# Autodesk Inventor assembly: Idler Right
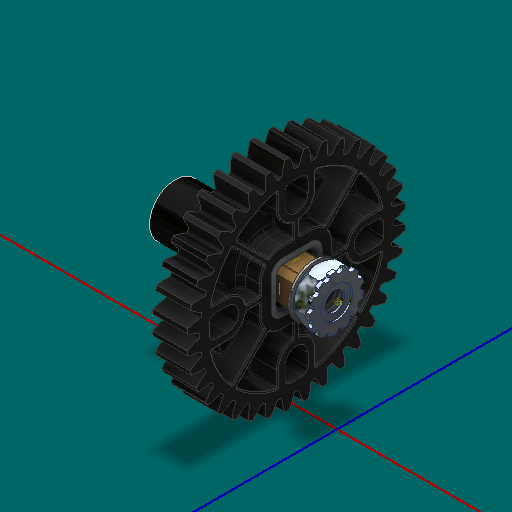
[picture p0: Inventor's stored thumbnail of the model, 512x512]
Saved by Autodesk Inventor 2025 (Build 290162000, 162)
## iProperties
Created: 2024-10-18
Part Number: Idler Right
Document SubType Name: Assembly
Designer: Averey Ku
Author: averey
## Documents named in this file (8)
- C:\Users\avere\VEX\High Stakes\CAD\V2\Chassis\Drivebay Right\Idler Right.iam
- C:\Users\avere\VEX\High Stakes\CAD\V2\Chassis\Drivebay Right\Half Cut HS 36T Gear, No Insert Right.ipt
- C:\Users\avere\VEX\High Stakes\CAD\V2\Chassis\Drivebay Right\HS Shaft Adapter Circle Right.ipt
- C:\Users\avere\VEX\High Stakes\CAD\V2\Chassis\Drivebay Right\Nut Keps Right2.ipt
- C:\Users\avere\VEX\High Stakes\CAD\ROBOPROS-CAD-Inventor\Motion\Spacers\Washer Steel\SWasher .375 OD x .015625.ipt
- D:\vex_robotics_high_stakes\hardware\cad\robpros_cad_lib\Motion\Spacers\Washer Steel.ipt
- C:\Users\avere\VEX\High Stakes\CAD\ROBOPROS-CAD-Inventor\Motion\Spacers\Spacer Nylon .375 OD\NSpacer .375 OD x .500.ipt
- C:\Users\avere\VEX\High Stakes\CAD\ROBOPROS-CAD-Inventor\Motion\Spacers\Spacer Nylon .375 OD.ipt
## Components (5 placed, 5 different names)
1. Half Cut HS 36T Gear, No Insert Right:1 — Insert:1, Angle:1, Insert:2
2. HS Shaft Adapter Circle Right:1 — Insert:1, Angle:1, Insert:3
3. Nut Keps Right2:1 — Mate:1, Insert:4
4. SWasher .375 OD x .015625:1 — Insert:2, Insert:4
5. NSpacer .375 OD x .500:1 — Insert:3
## Relationships (6: Insert 4, Angle 1, Mate 1)
- Insert:1 (-3.175 mm): Half Cut HS 36T Gear, No Insert Right:1 ↔ HS Shaft Adapter Circle Right:1
- Angle:1 (0 deg): Half Cut HS 36T Gear, No Insert Right:1 ↔ HS Shaft Adapter Circle Right:1
- Mate:1: Nut Keps Right2:1
- Insert:2 (3.175 mm): Half Cut HS 36T Gear, No Insert Right:1 ↔ SWasher .375 OD x .015625:1
- Insert:4: Nut Keps Right2:1 ↔ SWasher .375 OD x .015625:1
- Insert:3: HS Shaft Adapter Circle Right:1 ↔ NSpacer .375 OD x .500:1
